# Autodesk Inventor assembly: YAxisIdlerRight
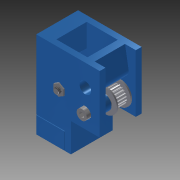
[picture p0: Inventor's stored thumbnail of the model, 180x180]
Saved by Autodesk Inventor 2015 SP1 (Build 190203100, 203)
## iProperties
Created: 2014-08-16
Part Number: YAxisIdlerRight
Document SubType Name: Assembly
Designer: Jack
Mass: 54.9534 g
Surface Area: 257.859 cm^2
Volume: 35.9784 cm^3
Density: 1.5274 g/cm^3
Author: Jack
Title: Y Idler Right
## Documents named in this file (11)
- C:\Users\Jack\ownCloud\Projects\CrossBot\InventorModel\YAxis\YAxisIdlerRight.iam
- C:\Users\Jack\ownCloud\Projects\CrossBot\InventorModel\YAxis\YAxisIdler\YIdlerCapRight.ipt
- C:\Users\Jack\ownCloud\Projects\CrossBot\InventorModel\Hardware\Bolts\SHCS\SHCS4\SHCS4x30.ipt
- C:\Users\Jack\ownCloud\Projects\CrossBot\InventorModel\Hardware\Nuts\Nut4.ipt
- C:\Users\Jack\ownCloud\Projects\CrossBot\InventorModel\Hardware\Bolts\SHCS\SHCS4\SHCS4x15.ipt
- C:\Users\Jack\ownCloud\Projects\CrossBot\InventorModel\Hardware\Wahsers\M4Washer.ipt
- C:\Users\Jack\ownCloud\Projects\CrossBot\InventorModel\Hardware\Belt\GT2Idler.iam
- C:\Users\Jack\ownCloud\Projects\CrossBot\InventorModel\YAxis\YAxisBeltIdlerSpacer.ipt
- C:\Users\Jack\ownCloud\Projects\CrossBot\InventorModel\Hardware\Bolts\FHS\FHS4\FHS4x8.ipt
- C:\Users\Jack\ownCloud\Projects\CrossBot\InventorModel\Hardware\Bolts\SHCS\SHCS4\SHCS4x8.ipt
- C:\Users\Jack\ownCloud\Projects\CrossBot\InventorModel\YAxis\YAxisIdler\YIdlerBlockRight.ipt
## Components (21 placed, 10 different names)
1. YIdlerCapRight:1 — Mate:18, Mate:15, Mate:17, Mate:16, Mate:77
2. M4Washer:1 — Mate:58, Mate:81, Mate:82
3. M4Washer:2 — Mate:35, Mate:60, Mate:85
4. M4Washer:3 — Mate:36, Mate:65, Mate:83
5. M4Washer:4 — Mate:64, Mate:80, Mate:84
6. GT2Idler:1 [sub-assembly] — Mate:50, Mate:82, Mate:85
7. GT2Idler:2 [sub-assembly] — Mate:54, Mate:83, Mate:84
8. YAxisBeltIdlerSpacer:1 — Mate:59, Mate:60
9. YAxisBeltIdlerSpacer:2 — Mate:61, Mate:65
10. YIdlerBlockRight:1 — Mate:62, Mate:63, Mate:66, Mate:67, Mate:68, Mate:69, Mate:71, Mate:72, Mate:73, Mate:74, Angle:1, Angle:2, Mate:75, Mate:76, Mate:77, Mate:78, Mate:79, Flush:1, Flush:2, Mate:80, Mate:81, Angle:3, Angle:4
11. SHCS4x30:2 — Mate:13, Mate:35, Mate:50, Mate:58, Mate:59, Mate:66, Mate:67
12. Nut4:2 — Mate:13, Mate:73, Angle:2
13. SHCS4x30:1 — Mate:11, Mate:36, Mate:54, Mate:61, Mate:64, Mate:68, Mate:69
14. Nut4:1 — Mate:11, Mate:74, Angle:1
15. FHS4x8:2 — Mate:79, Flush:1
16. SHCS4x8:1 — Mate:71, Mate:72
17. FHS4x8:1 — Mate:78, Flush:2
18. SHCS4x15:1 — Mate:18, Mate:15, Mate:19, Mate:75
19. SHCS4x15:2 — Mate:17, Mate:16, Mate:20, Mate:76
20. Nut4:3 — Mate:19, Mate:62, Angle:4
21. Nut4:4 — Mate:20, Mate:63, Angle:3
## Relationships (45: Mate 39, Angle 4, Flush 2)
- Mate:11: SHCS4x30:1 ↔ Nut4:1
- Mate:13: SHCS4x30:2 ↔ Nut4:2
- Mate:18: YIdlerCapRight:1 ↔ SHCS4x15:1
- Mate:15: YIdlerCapRight:1 ↔ SHCS4x15:1
- Mate:17: YIdlerCapRight:1 ↔ SHCS4x15:2
- Mate:16: YIdlerCapRight:1 ↔ SHCS4x15:2
- Mate:19: SHCS4x15:1 ↔ Nut4:3
- Mate:20: SHCS4x15:2 ↔ Nut4:4
- Mate:35: M4Washer:2 ↔ SHCS4x30:2
- Mate:36: M4Washer:3 ↔ SHCS4x30:1
- Mate:50: GT2Idler:1 ↔ SHCS4x30:2
- Mate:54: GT2Idler:2 ↔ SHCS4x30:1
- Mate:58: M4Washer:1 ↔ SHCS4x30:2
- Mate:59: YAxisBeltIdlerSpacer:1 ↔ SHCS4x30:2
- Mate:60: M4Washer:2 ↔ YAxisBeltIdlerSpacer:1
- Mate:61: YAxisBeltIdlerSpacer:2 ↔ SHCS4x30:1
- Mate:62: YIdlerBlockRight:1 ↔ Nut4:3
- Mate:63: YIdlerBlockRight:1 ↔ Nut4:4
- Mate:64: M4Washer:4 ↔ SHCS4x30:1
- Mate:65: M4Washer:3 ↔ YAxisBeltIdlerSpacer:2
- Mate:66: YIdlerBlockRight:1 ↔ SHCS4x30:2
- Mate:67: YIdlerBlockRight:1 ↔ SHCS4x30:2
- Mate:68: YIdlerBlockRight:1 ↔ SHCS4x30:1
- Mate:69: YIdlerBlockRight:1 ↔ SHCS4x30:1
- Mate:71: YIdlerBlockRight:1 ↔ SHCS4x8:1
- Mate:72: YIdlerBlockRight:1 ↔ SHCS4x8:1
- Mate:73: YIdlerBlockRight:1 ↔ Nut4:2
- Mate:74: YIdlerBlockRight:1 ↔ Nut4:1
- Angle:1 (0 deg): YIdlerBlockRight:1 ↔ Nut4:1
- Angle:2 (0 deg): YIdlerBlockRight:1 ↔ Nut4:2
- Mate:75: YIdlerBlockRight:1 ↔ SHCS4x15:1
- Mate:76: YIdlerBlockRight:1 ↔ SHCS4x15:2
- Mate:77: YIdlerCapRight:1 ↔ YIdlerBlockRight:1
- Mate:78: YIdlerBlockRight:1 ↔ FHS4x8:1
- Mate:79: YIdlerBlockRight:1 ↔ FHS4x8:2
- Flush:1: YIdlerBlockRight:1 ↔ FHS4x8:2
- Flush:2: YIdlerBlockRight:1 ↔ FHS4x8:1
- Mate:80: M4Washer:4 ↔ YIdlerBlockRight:1
- Mate:81: M4Washer:1 ↔ YIdlerBlockRight:1
- Mate:82: M4Washer:1 ↔ GT2Idler:1
- Mate:83: M4Washer:3 ↔ GT2Idler:2
- Mate:84: M4Washer:4 ↔ GT2Idler:2
- Mate:85: M4Washer:2 ↔ GT2Idler:1
- Angle:3 (0 deg): YIdlerBlockRight:1 ↔ Nut4:4
- Angle:4 (0 deg): YIdlerBlockRight:1 ↔ Nut4:3
